# Autodesk Inventor assembly: Montagem1
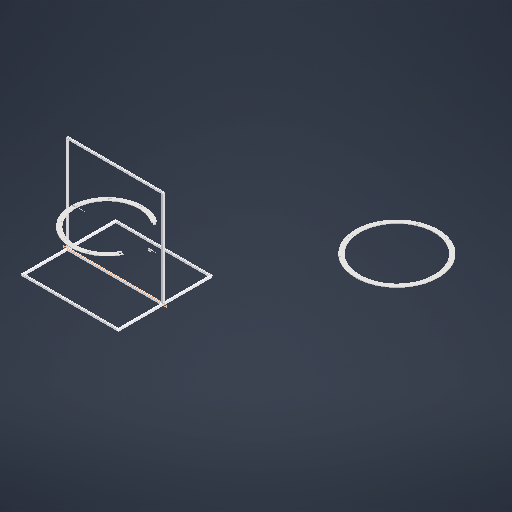
[picture p0: Inventor's stored thumbnail of the model, 512x512]
Saved by Autodesk Inventor 2026.2 (Build 302298000, 298)
## iProperties
Created: 2026-02-14
Part Number: Montagem1
Document SubType Name: Assembly
Designer: Ian
Author: Ian
## Documents named in this file (8)
- C:\Users\Ian\Desktop\MEUDRONE\Drone\BaseTestes 2.0\Montagem1.iam
- C:\Users\Ian\Desktop\MEUDRONE\Drone\BaseTestes 2.0\base.ipt
- C:\Users\Ian\Desktop\MEUDRONE\Drone\BaseTestes 2.0\baseExterna.ipt
- C:\Users\Ian\Desktop\MEUDRONE\Drone\BaseTestes 2.0\Apoio\barra 1,05m.ipt
- C:\Users\Ian\Desktop\MEUDRONE\Drone\BaseTestes 2.0\Apoio\barra 1,04.ipt
- C:\Users\Ian\Desktop\MEUDRONE\Drone\BaseTestes 2.0\Apoio\barra 1,08.ipt
- C:\Users\Ian\Desktop\MEUDRONE\Drone\BaseTestes 2.0\encaixeBase.ipt
- C:\Users\Ian\Desktop\MEUDRONE\Drone\BaseTestes 2.0\Eixo.ipt
## Components (28 placed, 7 different names)
1. base:1 — Alinhado:33, Coincidente:1, Coincidente:2
2. base:2 — Alinhado:33, Coincidente:1, Coincidente:2, Alinhado:36, Coincidente:7, Coincidente:8
3. base:3 — Alinhado:36, Coincidente:7, Coincidente:8
4. base:4 — Coincidente:15, Alinhado:40, Coincidente:16, Coincidente:47
5. base:5 — Coincidente:15, Alinhado:40, Coincidente:16, Coincidente:50
6. base:6 — Coincidente:46
7. base:7
8. barra 1,05m:1 — Coincidente:35, Alinhado:48, Alinhado:49, Coincidente:36, Alinhado:50, Alinhado:51, Coincidente:41, Alinhado:62, Coincidente:42, Coincidente:43, Alinhado:63, Alinhado:64
9. barra 1,04:1 — Coincidente:32, Coincidente:33, Coincidente:34, Coincidente:35, Alinhado:48, Alinhado:49, Alinhado:69
10. barra 1,04:2 — Coincidente:36, Alinhado:50, Alinhado:51, Coincidente:37, Alinhado:52, Alinhado:53
11. barra 1,05m:2 — Coincidente:37, Alinhado:52, Alinhado:53, Coincidente:44, Alinhado:65, Alinhado:66
12. barra 1,04:3 — Coincidente:41, Alinhado:62, Coincidente:42
13. barra 1,05m:1 — Coincidente:43, Alinhado:63, Alinhado:64
14. barra 1,05m:2 — Coincidente:44, Alinhado:65, Alinhado:66, Alinhado:67, Alinhado:68, Coincidente:45
15. barra 1,08:1 — Alinhado:67, Alinhado:68, Coincidente:45
16. encaixeBase:1 — Coincidente:47, Coincidente:49, Coincidente:50, Coincidente:54
17. encaixeBase:2 — Coincidente:52, Coincidente:55
18. Eixo:1 — Coincidente:54
19. Eixo:2 — Coincidente:55
20. baseExterna:1 — Coincidente:56, Alinhado:70, Coincidente:57, Alinhado:76
21. baseExterna:2 — Coincidente:56, Alinhado:70, Coincidente:57, Coincidente:60, Alinhado:72, Coincidente:61
22. baseExterna:3 — Coincidente:60, Alinhado:72, Coincidente:61
23. baseExterna:4 — Coincidente:68, Coincidente:69
24. baseExterna:5 — Alinhado:76, Coincidente:68, Coincidente:69
25. baseExterna:6
26. baseExterna:7 — Coincidente:70, Coincidente:71, Alinhado:77
27. baseExterna:8 — Coincidente:70, Coincidente:71, Alinhado:77, Alinhado:78, Coincidente:72, Coincidente:73
28. baseExterna:9 — Alinhado:78, Coincidente:72, Coincidente:73
## Relationships (75: Mate 46, Flush 29)
- Alinhado:32 [Flush] (455 mm)
- Alinhado:33 [Flush]: base:1 ↔ base:2
- Coincidente:1 [Mate]: base:1 ↔ base:2
- Coincidente:2 [Mate]: base:1 ↔ base:2
- [Flush]: base:3 ↔ base:4
- [Mate]: base:3 ↔ base:4
- [Mate]: base:3 ↔ base:4
- Alinhado:36 [Flush]: base:2 ↔ base:3
- Coincidente:7 [Mate]: base:2 ↔ base:3
- Coincidente:8 [Mate]: base:2 ↔ base:3
- [Flush]: base:5 ↔ base:6
- [Mate]: base:5 ↔ base:6
- [Mate]: base:5 ↔ base:6
- [Flush]: base:6 ↔ base:7
- [Mate]: base:6 ↔ base:7
- [Mate]: base:6 ↔ base:7
- Coincidente:15 [Mate]: base:4 ↔ base:5
- Alinhado:40 [Flush]: base:4 ↔ base:5
- Coincidente:16 [Mate]: base:4 ↔ base:5
- Coincidente:32 [Mate]: barra 1,04:1
- Coincidente:33 [Mate]: barra 1,04:1
- Coincidente:34 [Mate]: barra 1,04:1
- Coincidente:35 [Mate]: barra 1,05m:1 ↔ barra 1,04:1
- Alinhado:48 [Flush]: barra 1,05m:1 ↔ barra 1,04:1
- Alinhado:49 [Flush]: barra 1,05m:1 ↔ barra 1,04:1
- Coincidente:36 [Mate]: barra 1,05m:1 ↔ barra 1,04:2
- Alinhado:50 [Flush]: barra 1,05m:1 ↔ barra 1,04:2
- Alinhado:51 [Flush]: barra 1,05m:1 ↔ barra 1,04:2
- Coincidente:37 [Mate]: barra 1,04:2 ↔ barra 1,05m:2
- Alinhado:52 [Flush]: barra 1,04:2 ↔ barra 1,05m:2
- Alinhado:53 [Flush]: barra 1,04:2 ↔ barra 1,05m:2
- Coincidente:41 [Mate] (-555 mm): barra 1,05m:1 ↔ barra 1,04:3
- Alinhado:62 [Flush]: barra 1,05m:1 ↔ barra 1,04:3
- Coincidente:42 [Mate]: barra 1,05m:1 ↔ barra 1,04:3
- Coincidente:43 [Mate]: barra 1,05m:1
- Alinhado:63 [Flush]: barra 1,05m:1
- Alinhado:64 [Flush] (535 mm): barra 1,05m:1
- Coincidente:44 [Mate]: barra 1,05m:2
- Alinhado:65 [Flush] (535 mm): barra 1,05m:2
- Alinhado:66 [Flush]: barra 1,05m:2
- Alinhado:67 [Flush]: barra 1,05m:2 ↔ barra 1,08:1
- Alinhado:68 [Flush]: barra 1,05m:2 ↔ barra 1,08:1
- Coincidente:45 [Mate]: barra 1,05m:2 ↔ barra 1,08:1
- Coincidente:46 [Mate] (450 mm): base:6
- Coincidente:47 [Mate]: base:4 ↔ encaixeBase:1
- Alinhado:69 [Flush] (-505 mm): barra 1,04:1
- Coincidente:49 [Mate]: encaixeBase:1
- Coincidente:50 [Mate] (10 mm): base:5 ↔ encaixeBase:1
- Coincidente:52 [Mate]: encaixeBase:2
- Coincidente:54 [Mate]: encaixeBase:1 ↔ Eixo:1
- Coincidente:55 [Mate]: encaixeBase:2 ↔ Eixo:2
- Coincidente:56 [Mate]: baseExterna:1 ↔ baseExterna:2
- Alinhado:70 [Flush]: baseExterna:1 ↔ baseExterna:2
- Coincidente:57 [Mate]: baseExterna:1 ↔ baseExterna:2
- [Mate]: baseExterna:3 ↔ baseExterna:4
- [Flush]: baseExterna:3 ↔ baseExterna:4
- [Mate]: baseExterna:3 ↔ baseExterna:4
- Coincidente:60 [Mate]: baseExterna:2 ↔ baseExterna:3
- Alinhado:72 [Flush]: baseExterna:2 ↔ baseExterna:3
- Coincidente:61 [Mate]: baseExterna:2 ↔ baseExterna:3
- [Mate]: baseExterna:5 ↔ baseExterna:6
- [Flush]: baseExterna:5 ↔ baseExterna:6
- [Mate]: baseExterna:5 ↔ baseExterna:6
- [Mate]: baseExterna:6 ↔ baseExterna:7
- [Flush]: baseExterna:6 ↔ baseExterna:7
- [Mate]: baseExterna:6 ↔ baseExterna:7
- Alinhado:76 [Flush]: baseExterna:1 ↔ baseExterna:5
- Coincidente:68 [Mate]: baseExterna:4 ↔ baseExterna:5
- Coincidente:69 [Mate]: baseExterna:4 ↔ baseExterna:5
- Coincidente:70 [Mate]: baseExterna:7 ↔ baseExterna:8
- Coincidente:71 [Mate]: baseExterna:7 ↔ baseExterna:8
- Alinhado:77 [Flush]: baseExterna:7 ↔ baseExterna:8
- Alinhado:78 [Flush]: baseExterna:8 ↔ baseExterna:9
- Coincidente:72 [Mate]: baseExterna:8 ↔ baseExterna:9
- Coincidente:73 [Mate]: baseExterna:8 ↔ baseExterna:9
## Named parameters: d221_d218 = 0 mm, d222_d219 = 0 mm, d223_d220 = 0 mm, d230_d227 = 0 mm, d231_d228 = 0 mm, d232_d229 = 0 mm, d233_d218 = 0 mm, d234_d219 = 0 mm, d235_d220 = 0 mm, d323_d320 = 0 mm, d324_d321 = 0 mm, d325_d322 = 0 mm, d329_d320 = 0 mm, d330_d321 = 0 mm, d331_d322 = 0 mm, d335_d326 = 0 mm, d336_d327 = 0 mm, d337_d328 = 0 mm
